# Autodesk Inventor assembly: test
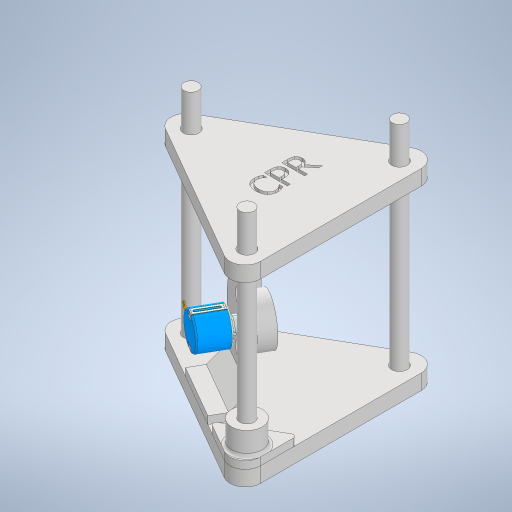
[picture p0: Inventor's stored thumbnail of the model, 512x512]
Saved by Autodesk Inventor 2023 (Build 270158000, 158)
## iProperties
Created: 2022-11-10
Part Number: test
Document SubType Name: Assembly
Designer: eahil
Author: eahil
## Documents named in this file (8)
- C:\Users\eahil\OneDrive - McMaster University\capstone\rig\Inventor_Model\test.iam
- C:\Users\eahil\OneDrive - McMaster University\capstone\rig\Inventor_Model\base.ipt
- C:\Users\eahil\OneDrive - McMaster University\capstone\rig\Inventor_Model\pinion.ipt
- C:\Users\eahil\OneDrive - McMaster University\capstone\rig\Inventor_Model\pot_stand.ipt
- C:\Users\eahil\OneDrive - McMaster University\capstone\rig\Inventor_Model\push_plate.ipt
- C:\Users\eahil\OneDrive - McMaster University\capstone\rig\Inventor_Model\rack.ipt
- C:\Users\eahil\OneDrive - McMaster University\capstone\rig\Inventor_Model\rod.ipt
- C:\Users\eahil\OneDrive - McMaster University\capstone\rig\Inventor_Model\3D_model_PN_3540s-1-503l.ipt
## Components (9 placed, 7 different names)
1. base:1 — Insert:1, Insert:2, Insert:3, Mate:3, Mate:4
2. pinion:1 — Mate:7, Mate:8, Tangent:1, Flush:1
3. pot_stand:1 — Mate:3, Mate:4, Mate:5, Angle:1, Angle:2, Mate:7, Mate:8
4. push_plate:1 — Mate:1, Mate:2, Mate:6
5. rack:1 — Mate:6, Tangent:1, Flush:1
6. rod:1 — Insert:2, Mate:1
7. rod:2 — Insert:3
8. rod:3 — Insert:1, Mate:2
9. 3D_model_PN_3540s-1-503l:1 — Mate:5, Angle:1, Angle:2
## Relationships (15: Mate 8, Insert 3, Angle 2, Tangent 1, Flush 1)
- Insert:1: base:1 ↔ rod:3
- Insert:2: base:1 ↔ rod:1
- Insert:3: base:1 ↔ rod:2
- Mate:1: push_plate:1 ↔ rod:1
- Mate:2: push_plate:1 ↔ rod:3
- Mate:3: base:1 ↔ pot_stand:1
- Mate:4: base:1 ↔ pot_stand:1
- Mate:5: pot_stand:1 ↔ 3D_model_PN_3540s-1-503l:1
- Angle:1 (0 deg): pot_stand:1 ↔ 3D_model_PN_3540s-1-503l:1
- Angle:2 (0 deg): pot_stand:1 ↔ 3D_model_PN_3540s-1-503l:1
- Mate:6: push_plate:1 ↔ rack:1
- Mate:7: pinion:1 ↔ pot_stand:1
- Mate:8 (2 mm): pinion:1 ↔ pot_stand:1
- Tangent:1: pinion:1 ↔ rack:1
- Flush:1: pinion:1 ↔ rack:1
